# Autodesk Inventor assembly: EvelMidFrame
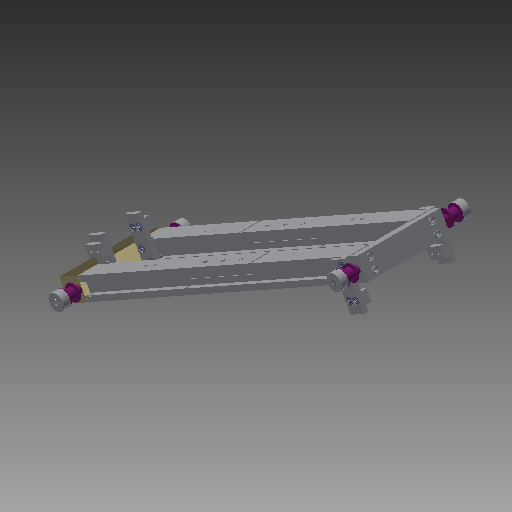
[picture p0: Inventor's stored thumbnail of the model, 512x512]
Saved by Autodesk Inventor 2019 (Build 230136000, 136)
## iProperties
Created: 2019-09-29
Part Number: EvelMidFrame
Document SubType Name: Assembly
Designer: james
Author: james
## Documents named in this file (5)
- F:\JimsDesign\Jims2020FTC\EvelMidFrame.iam
- F:\JimsDesign\Jims2020FTC\ElevatorFrame.iam
- F:\JimsDesign\Jims2020FTC\FullElevatorShart.iam
- F:\JimsDesign\Jims2020FTC\SliderLeft.iam
- F:\JimsDesign\Jims2020FTC\SliderRight.iam
## Components (7 placed, 4 different names)
1. ElevatorFrame:1 [sub-assembly] — Mate:2, Mate:17, Mate:18, Mate:19, Mate:20, Mate:21, Mate:22, Mate:26, Mate:27, Mate:28, Mate:29, Mate:30, Mate:31, Mate:32, Mate:33, Mate:34
2. FullElevatorShart:1 [sub-assembly] — Mate:17, Mate:19
3. FullElevatorShart:2 [sub-assembly] — Mate:2, Mate:18
4. SliderRight:1 [sub-assembly] — Mate:20, Mate:21, Mate:22
5. SliderRight:3 [sub-assembly] — Mate:26, Mate:27, Mate:28
6. SliderLeft:1 [sub-assembly] — Mate:32, Mate:33, Mate:34
7. SliderLeft:2 [sub-assembly] — Mate:29, Mate:30, Mate:31
## Relationships (16: Mate 16)
- Mate:2: ElevatorFrame:1 ↔ FullElevatorShart:2
- Mate:17: ElevatorFrame:1 ↔ FullElevatorShart:1
- Mate:18: ElevatorFrame:1 ↔ FullElevatorShart:2
- Mate:19: ElevatorFrame:1 ↔ FullElevatorShart:1
- Mate:20: ElevatorFrame:1 ↔ SliderRight:1
- Mate:21: ElevatorFrame:1 ↔ SliderRight:1
- Mate:22: ElevatorFrame:1 ↔ SliderRight:1
- Mate:26: ElevatorFrame:1 ↔ SliderRight:3
- Mate:27: ElevatorFrame:1 ↔ SliderRight:3
- Mate:28: ElevatorFrame:1 ↔ SliderRight:3
- Mate:29: ElevatorFrame:1 ↔ SliderLeft:2
- Mate:30: ElevatorFrame:1 ↔ SliderLeft:2
- Mate:31: ElevatorFrame:1 ↔ SliderLeft:2
- Mate:32: ElevatorFrame:1 ↔ SliderLeft:1
- Mate:33: ElevatorFrame:1 ↔ SliderLeft:1
- Mate:34: ElevatorFrame:1 ↔ SliderLeft:1
